# Autodesk Inventor assembly: FGR AL-2-PGN-plus-P 160,PGN-plus-P 160-2-AS-P1Aluminium86.5165110452001216049.500000000000000002
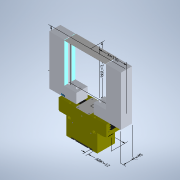
[picture p0: Inventor's stored thumbnail of the model, 180x180]
Saved by Autodesk Inventor 2021 (Build 250183000, 183)
## iProperties
Category: PARTsolutions
Company: SCHUNK
Created: 2025-07-30
Part Number: FGR AL-2-PGN-plus-P 160,PGN-plus-P 160-2-AS-P1Aluminium86.5165110452001216049.500000000000000002
Catalog Web Link: www.cadenas.de
Description: FGR-Customizable gripper fingers
Vendor: SCHUNK
Document SubType Name: Assembly
Designer: psAdmin
Manufacturer: SCHUNK
Mass: 2444.6 g
Surface Area: 3300.31 cm^2
Volume: 2444.6 cm^3
Density: 1 g/cm^3
Title: FGR AL-2-PGN-plus-P 160, 11045200SPANNKONT.
Author: Cadenas PARTsolutions
Comments: Customizable gripper fingers
PSOL_IDENT_0: {$CADENAS_DATA/23d-libs/schunk/greifsysteme/konfigurationen/system_baukasten/easy_finger/easy_finger
PSOL_IDENT_1: _asm_at.prj},511 {M=Nenngewinde},{VTYP=3D},{STYP=ASSTAB},{NB=FGR AL-2-PGN-plus-P 160,PGN-plus-P 160-
PSOL_IDENT_2: 2-AS-P1Aluminium86.5165110452001216049.500000000000000002},{LINA=FGR AL-2-PGN-plus-P 160, 11045200SP
PSOL_IDENT_3: ANNKONT.},{NN=FGR},{DATE=29.07.2025 14:42:42},{GEOMDATE=25.10.2024 10:48:57},{VERSION=},{LINEID=10},
PSOL_IDENT_4: {WBVAR=BR,BGVR,ASIS,SPANNKONT,CNSMAT,WAERMEBE,HUB,RH,X,Y,Z,DWS,ABK,GFL,GFT,PP,PW,RA,EFO,FASE1,FL1,FA
PSOL_IDENT_5: SE2,FL2,FASE3,FW3,FL3,FASE4,FW4,FL4,BM},{WBNUMERIC=HUB,RH,X,Y,Z,DWS,ABK,GFL,GFT,PP,PW,RA,EFO,FL1,FL2
PSOL_IDENT_6: ,FASE3,FW3,FL3,FW4,FL4,BM}  {NB=FGR AL-2-PGN-plus-P 160,PGN-plus-P 160-2-AS-P1Aluminium86.5165110452
PSOL_IDENT_7: 001216049.500000000000000002},{LINA=FGR AL-2-PGN-plus-P 160, 11045200SPANNKONT.},{KT=DUMMY},{NT=Kund
PSOL_IDENT_8: enspezifisch konfigurierbare Greiferfinger},{START=Geometriemodell 2},{VERSION=1},{VER=V1},{MATN=378
PSOL_IDENT_9: 6171200_fgr_gl_ia_v1},{XMLMATN=material|},{XMLMAT=AlZn55MgCu_EN-AW-7075_34365},{TYP=FGR AL-2-PGN-plu
PSOL_IDENT_10: s-P 160},{TYPX=PGN-plus-P 160},{TYPXMAT=AL},{TYPXX=PGN-plus-P 160},{BR=PGN-plus-P},{BG=160.0},{BGVR=
PSOL_IDENT_11: PGN-plus-P 160-2-AS-P},{BGVRX='PGN-plus-P 40','PGN-plus-P 40','PGN-plus-P 40-SD','PGN-plus-P 40-SD','
PSOL_IDENT_12: PGN-plus-P 40-K','PGN-plus-P 40-K','PGN-plus-P 40-V','PGN-plus-P 40-V','PGN-plus-P 40-P','PGN-plus-P
PSOL_IDENT_13: 40-P','PGN-plus-P 40-AS','PGN-plus-P 40-AS','PGN-plus-P 40-AS-SD','PGN-plus-P 40-AS-SD','PGN-plus-P
PSOL_IDENT_14: 40-AS-K','PGN-plus-P 40-AS-K','PGN-plus-P 40-AS-V','PGN-plus-P 40-AS-V','PGN-plus-P 40-AS-P','PGN-p
PSOL_IDENT_15: lus-P 40-AS-P','PGN-plus-P 40-IS','PGN-plus-P 40-IS','PGN-plus-P 40-IS-SD','PGN-plus-P 40-IS-SD','PG
PSOL_IDENT_16: N-plus-P 40-IS-K','PGN-plus-P 40-IS-K','PGN-plus-P 40-IS-V','PGN-plus-P 40-IS-V','PGN-plus-P 50-1','
PSOL_IDENT_17: PGN-plus-P 50-1','PGN-plus-P 50-1-SD','PGN-plus-P 50-1-SD','PGN-plus-P 50-1-K','PGN-plus-P 50-1-K','
PSOL_IDENT_18: PGN-plus-P 50-1-V','PGN-plus-P 50-1-V','PGN-plus-P 50-1-P','PGN-plus-P 50-1-P','PGN-plus-P 50-2','PG
PSOL_IDENT_19: N-plus-P 50-2','PGN-plus-P 50-2-SD','PGN-plus-P 50-2-SD','PGN-plus-P 50-2-K','PGN-plus-P 50-2-K','PG
PSOL_IDENT_20: N-plus-P 50-2-V','PGN-plus-P 50-2-V','PGN-plus-P 50-2-P','PGN-plus-P 50-2-P','PGN-plus-P 50-1-AS','P
PSOL_IDENT_21: GN-plus-P 50-1-AS','PGN-plus-P 50-1-AS-SD','PGN-plus-P 50-1-AS-SD','PGN-plus-P 50-1-AS-K','PGN-plus-
PSOL_IDENT_22: P 50-1-AS-K','PGN-plus-P 50-1-AS-V','PGN-plus-P 50-1-AS-V','PGN-plus-P 50-1-AS-P','PGN-plus-P 50-1-A
PSOL_IDENT_23: S-P','PGN-plus-P 50-2-AS','PGN-plus-P 50-2-AS','PGN-plus-P 50-2-AS-SD','PGN-plus-P 50-2-AS-SD','PGN-
PSOL_IDENT_24: plus-P 50-2-AS-K','PGN-plus-P 50-2-AS-K','PGN-plus-P 50-2-AS-V','PGN-plus-P 50-2-AS-V','PGN-plus-P 5
PSOL_IDENT_25: 0-2-AS-P','PGN-plus-P 50-2-AS-P','PGN-plus-P 50-1-IS','PGN-plus-P 50-1-IS','PGN-plus-P 50-1-IS-SD','
PSOL_IDENT_26: PGN-plus-P 50-1-IS-SD','PGN-plus-P 50-1-IS-K','PGN-plus-P 50-1-IS-K','PGN-plus-P 50-1-IS-V','PGN-plu
PSOL_IDENT_27: s-P 50-1-IS-V','PGN-plus-P 50-2-IS','PGN-plus-P 50-2-IS','PGN-plus-P 50-2-IS-SD','PGN-plus-P 50-2-IS
PSOL_IDENT_28: -SD','PGN-plus-P 50-2-IS-K','PGN-plus-P 50-2-IS-K','PGN-plus-P 50-2-IS-V','PGN-plus-P 50-2-IS-V','PG
PSOL_IDENT_29: N-plus-P 64-1','PGN-plus-P 64-1','PGN-plus-P 64-1-SD','PGN-plus-P 64-1-SD','PGN-plus-P 64-1-K','PGN-
PSOL_IDENT_30: plus-P 64-1-K','PGN-plus-P 64-1-V','PGN-plus-P 64-1-V','PGN-plus-P 64-1-P','PGN-plus-P 64-1-P','PGN-
PSOL_IDENT_31: plus-P 64-2','PGN-plus-P 64-2','PGN-plus-P 64-2-SD','PGN-plus-P 64-2-SD','PGN-plus-P 64-2-K','PGN-pl
PSOL_IDENT_32: us-P 64-2-K','PGN-plus-P 64-2-V','PGN-plus-P 64-2-V','PGN-plus-P 64-2-P','PGN-plus-P 64-2-P','PGN-pl
PSOL_IDENT_33: us-P 64-1-AS','PGN-plus-P 64-1-AS','PGN-plus-P 64-1-AS-SD','PGN-plus-P 64-1-AS-SD','PGN-plus-P 64-1-
PSOL_IDENT_34: AS-K','PGN-plus-P 64-1-AS-K','PGN-plus-P 64-1-AS-V','PGN-plus-P 64-1-AS-V','PGN-plus-P 64-1-AS-P','P
PSOL_IDENT_35: GN-plus-P 64-1-AS-P','PGN-plus-P 64-2-AS','PGN-plus-P 64-2-AS','PGN-plus-P 64-1-IS','PGN-plus-P 64-1
PSOL_IDENT_36: -IS','PGN-plus-P 64-1-IS-SD','PGN-plus-P 64-1-IS-SD','PGN-plus-P 64-1-IS-K','PGN-plus-P 64-1-IS-K','
PSOL_IDENT_37: PGN-plus-P 64-1-IS-V','PGN-plus-P 64-1-IS-V','PGN-plus-P 64-2-IS','PGN-plus-P 64-2-IS','PGN-plus-P 6
PSOL_IDENT_38: 4-2-IS-SD','PGN-plus-P 64-2-IS-SD','PGN-plus-P 64-2-IS-K','PGN-plus-P 64-2-IS-K','PGN-plus-P 64-2-V'
PSOL_IDENT_39: ,'PGN-plus-P 64-2-V','PGN-plus-P 80-1','PGN-plus-P 80-1','PGN-plus-P 80-1-SD','PGN-plus-P 80-1-SD','
PSOL_IDENT_40: PGN-plus-P 80-1-K','PGN-plus-P 80-1-K','PGN-plus-P 80-1-V','PGN-plus-P 80-1-V','PGN-plus-P 80-1-P','
PSOL_IDENT_41: PGN-plus-P 80-1-P','PGN-plus-P 80-2','PGN-plus-P 80-2','PGN-plus-P 80-2-SD','PGN-plus-P 80-2-SD','PG
PSOL_IDENT_42: N-plus-P 80-2-K','PGN-plus-P 80-2-K','PGN-plus-P 80-2-V','PGN-plus-P 80-2-V','PGN-plus-P 80-2-P','PG
PSOL_IDENT_43: N-plus-P 80-2-P','PGN-plus-P 80-1-AS','PGN-plus-P 80-1-AS','PGN-plus-P 80-1-AS-SD','PGN-plus-P 80-1-
PSOL_IDENT_44: AS-SD','PGN-plus-P 80-1-AS-K','PGN-plus-P 80-1-AS-K','PGN-plus-P 80-1-AS-V','PGN-plus-P 80-1-AS-V','
PSOL_IDENT_45: PGN-plus-P 80-1-AS-P','PGN-plus-P 80-1-AS-P','PGN-plus-P 80-2-AS','PGN-plus-P 80-2-AS','PGN-plus-P 8
PSOL_IDENT_46: 0-2-AS-SD', 'PGN-plus-P 80-2-AS-SD','PGN-plus-P 80-2-AS-K','PGN-plus-P 80-2-AS-K','PGN-plus-P 80-2-A
PSOL_IDENT_47: S-V','PGN-plus-P 80-2-AS-V','PGN-plus-P 80-2-AS-P','PGN-plus-P 80-2-AS-P','PGN-plus-P 80-1-IS','PGN-
PSOL_IDENT_48: plus-P 80-1-IS','PGN-plus-P 80-1-IS-SD','PGN-plus-P 80-1-IS-SD','PGN-plus-P 80-1-IS-K','PGN-plus-P 8
PSOL_IDENT_49: 0-1-IS-K','PGN-plus-P 80-1-IS-V','PGN-plus-P 80-1-IS-V','PGN-plus-P 80-2-IS','PGN-plus-P 80-2-IS','P
PSOL_IDENT_50: GN-plus-P 80-2-IS-SD','PGN-plus-P 80-2-IS-SD','PGN-plus-P 80-2-IS-K','PGN-plus-P 80-2-IS-K','PGN-plu
PSOL_IDENT_51: s-P 80-2-IS-V','PGN-plus-P 80-2-IS-V','PGN-plus-P 100-1','PGN-plus-P 100-1','PGN-plus-P 100-1-SD','P
PSOL_IDENT_52: GN-plus-P 100-1-SD','PGN-plus-P 100-1-K','PGN-plus-P 100-1-K','PGN-plus-P 100-1-V','PGN-plus-P 100-1
PSOL_IDENT_53: -V','PGN-plus-P 100-1-P','PGN-plus-P 100-1-P','PGN-plus-P 100-2','PGN-plus-P 100-2','PGN-plus-P 100-
PSOL_IDENT_54: 2-SD','PGN-plus-P 100-2-SD','PGN-plus-P 100-2-K','PGN-plus-P 100-2-K','PGN-plus-P 100-2-V','PGN-plus
PSOL_IDENT_55: -P 100-2-V','PGN-plus-P 100-2-P','PGN-plus-P 100-2-P','PGN-plus-P 100-1-AS','PGN-plus-P 100-1-AS','P
PSOL_IDENT_56: GN-plus-P 100-1-AS-SD','PGN-plus-P 100-1-AS-SD','PGN-plus-P 100-1-AS-K','PGN-plus-P 100-1-AS-K','PGN
PSOL_IDENT_57: -plus-P 100-1-AS-V','PGN-plus-P 100-1-AS-V','PGN-plus-P 100-1-AS-P','PGN-plus-P 100-1-AS-P','PGN-plu
PSOL_IDENT_58: s-P 100-2-AS','PGN-plus-P 100-2-AS','PGN-plus-P 100-2-AS-SD','PGN-plus-P 100-2-AS-SD','PGN-plus-P 10
PSOL_IDENT_59: 0-2-AS-K','PGN-plus-P 100-2-AS-K','PGN-plus-P 100-2-AS-V','PGN-plus-P 100-2-AS-V','PGN-plus-P 100-2-
PSOL_IDENT_60: AS-P','PGN-plus-P 100-2-AS-P','PGN-plus-P 100-1-IS','PGN-plus-P 100-1-IS','PGN-plus-P 100-1-IS-SD','
PSOL_IDENT_61: PGN-plus-P 100-1-IS-SD','PGN-plus-P 100-1-IS-K','PGN-plus-P 100-1-IS-K','PGN-plus-P 100-1-IS-V','PGN
PSOL_IDENT_62: -plus-P 100-1-IS-V','PGN-plus-P 100-2-IS','PGN-plus-P 100-2-IS','PGN-plus-P 100-2-IS-SD','PGN-plus-P
PSOL_IDENT_63: 100-2-IS-SD','PGN-plus-P 100-2-IS-K','PGN-plus-P 100-2-IS-K','PGN-plus-P 100-2-IS-V','PGN-plus-P 10
PSOL_IDENT_64: 0-2-IS-V','PGN-plus-P 125-1','PGN-plus-P 125-1','PGN-plus-P 125-1-SD','PGN-plus-P 125-1-SD','PGN-plu
PSOL_IDENT_65: s-P 125-1-K','PGN-plus-P 125-1-K','PGN-plus-P 125-1-V','PGN-plus-P 125-1-V','PGN-plus-P 125-1-P','PG
PSOL_IDENT_66: N-plus-P 125-1-P','PGN-plus-P 125-2','PGN-plus-P 125-2','PGN-plus-P 125-2-SD','PGN-plus-P 125-2-SD','
PSOL_IDENT_67: PGN-plus-P 125-2-K','PGN-plus-P 125-2-K','PGN-plus-P 125-2-V','PGN-plus-P 125-2-V','PGN-plus-P 125-2
PSOL_IDENT_68: -P','PGN-plus-P 125-2-P','PGN-plus-P 125-1-AS','PGN-plus-P 125-1-AS','PGN-plus-P 125-1-AS-SD','PGN-p
PSOL_IDENT_69: lus-P 125-1-AS-SD','PGN-plus-P 125-1-AS-K','PGN-plus-P 125-1-AS-K','PGN-plus-P 125-1-AS-V','PGN-plus
PSOL_IDENT_70: -P 125-1-AS-V','PGN-plus-P 125-1-AS-P','PGN-plus-P 125-1-AS-P','PGN-plus-P 125-2-AS','PGN-plus-P 125
PSOL_IDENT_71: -2-AS','PGN-plus-P 125-2-AS-SD','PGN-plus-P 125-2-AS-SD','PGN-plus-P 125-2-AS-K','PGN-plus-P 125-2-A
PSOL_IDENT_72: S-K','PGN-plus-P 125-2-AS-V','PGN-plus-P 125-2-AS-V','PGN-plus-P 125-2-AS-P','PGN-plus-P 125-2-AS-P'
PSOL_IDENT_73: ,'PGN-plus-P 125-1-IS','PGN-plus-P 125-1-IS','PGN-plus-P 125-1-IS-SD','PGN-plus-P 125-1-IS-SD','PGN-
PSOL_IDENT_74: plus-P 125-1-IS-K','PGN-plus-P 125-1-IS-K','PGN-plus-P 125-1-IS-V','PGN-plus-P 125-1-IS-V','PGN-plus
PSOL_IDENT_75: -P 125-2-IS','PGN-plus-P 125-2-IS','PGN-plus-P 125-2-IS-SD','PGN-plus-P 125-2-IS-SD','PGN-plus-P 125
PSOL_IDENT_76: -2-IS-K','PGN-plus-P 125-2-IS-K','PGN-plus-P 125-2-IS-V','PGN-plus-P 125-2-IS-V','PGN-plus-P 160-1','
PSOL_IDENT_77: PGN-plus-P 160-1','PGN-plus-P 160-1-SD','PGN-plus-P 160-1-SD','PGN-plus-P 160-1-K','PGN-plus-P 160-1
PSOL_IDENT_78: -K','PGN-plus-P 160-1-V','PGN-plus-P 160-1-V','PGN-plus-P 160-1-P','PGN-plus-P 160-1-P','PGN-plus-P
PSOL_IDENT_79: 160-2','PGN-plus-P 160-2','PGN-plus-P 160-2-SD','PGN-plus-P 160-2-SD','PGN-plus-P 160-2-K','PGN-plus
PSOL_IDENT_80: -P 160-2-K','PGN-plus-P 160-2-V','PGN-plus-P 160-2-V','PGN-plus-P 160-2-P','PGN-plus-P 160-2-P','PGN
PSOL_IDENT_81: -plus-P 160-1-AS','PGN-plus-P 160-1-AS','PGN-plus-P 160-1-AS-SD','PGN-plus-P 160-1-AS-SD','PGN-plus-
PSOL_IDENT_82: P 160-1-AS-K','PGN-plus-P 160-1-AS-K','PGN-plus-P 160-1-AS-V','PGN-plus-P 160-1-AS-V','PGN-plus-P 16
PSOL_IDENT_83: 0-1-AS-P','PGN-plus-P 160-1-AS-P','PGN-plus-P 160-2-AS','PGN-plus-P 160-2-AS','PGN-plus-P 160-2-AS-S
PSOL_IDENT_84: D','PGN-plus-P 160-2-AS-SD','PGN-plus-P 160-2-AS-K','PGN-plus-P 160-2-AS-K','PGN-plus-P 160-2-AS-V','
PSOL_IDENT_85: PGN-plus-P 160-2-AS-V','PGN-plus-P 160-2-AS-P','PGN-plus-P 160-2-AS-P','PGN-plus-P 160-1-IS','PGN-pl
PSOL_IDENT_86: us-P 160-1-IS','PGN-plus-P 160-1-IS-SD','PGN-plus-P 160-1-IS-SD','PGN-plus-P 160-1-IS-K','PGN-plus-P
PSOL_IDENT_87: 160-1-IS-K','PGN-plus-P 160-1-IS-V','PGN-plus-P 160-1-IS-V','PGN-plus-P 160-2-IS','PGN-plus-P 160-2
PSOL_IDENT_88: -IS','PGN-plus-P 160-2-IS-SD','PGN-plus-P 160-2-IS-SD','PGN-plus-P 160-2-IS-K','PGN-plus-P 160-2-IS-
PSOL_IDENT_89: K','PGN-plus-P 160-2-IS-V','PGN-plus-P 160-2-IS-V','PGN-plus-P 200-1','PGN-plus-P 200-1','PGN-plus-P
PSOL_IDENT_90: 200-1-SD','PGN-plus-P 200-1-SD','PGN-plus-P 200-1-K','PGN-plus-P 200-1-K','PGN-plus-P 200-1-V','PGN
PSOL_IDENT_91: -plus-P 200-1-V','PGN-plus-P 200-1-P','PGN-plus-P 200-1-P','PGN-plus-P 200-2','PGN-plus-P 200-2','PG
PSOL_IDENT_92: N-plus-P 200-2-SD','PGN-plus-P 200-2-SD','PGN-plus-P 200-2-K','PGN-plus-P 200-2-K','PGN-plus-P 200-2
PSOL_IDENT_93: -V','PGN-plus-P 200-2-V','PGN-plus-P 200-2-P','PGN-plus-P 200-2-P','PGN-plus-P 200-1-AS','PGN-plus-P
PSOL_IDENT_94: 200-1-AS','PGN-plus-P 200-1-AS-SD','PGN-plus-P 200-1-AS-SD','PGN-plus-P 200-1-AS-K','PGN-plus-P 200
PSOL_IDENT_95: -1-AS-K','PGN-plus-P 200-1-AS-V','PGN-plus-P 200-1-AS-V','PGN-plus-P 200-1-AS-P','PGN-plus-P 200-1-A
PSOL_IDENT_96: S-P','PGN-plus-P 200-2-AS','PGN-plus-P 200-2-AS','PGN-plus-P 200-2-AS-SD','PGN-plus-P 200-2-AS-SD','
PSOL_IDENT_97: PGN-plus-P 200-2-AS-K','PGN-plus-P 200-2-AS-K','PGN-plus-P 200-2-AS-V','PGN-plus-P 200-2-AS-V','PGN-
PSOL_IDENT_98: plus-P 200-2-AS-P','PGN-plus-P 200-2-AS-P','PGN-plus-P 200-1-IS','PGN-plus-P 200-1-IS','PGN-plus-P 2
PSOL_IDENT_99: 00-1-IS-SD','PGN-plus-P 200-1-IS-SD','PGN-plus-P 200-1-IS-K','PGN-plus-P 200-1-IS-K','PGN-plus-P 200
PSOL_IDENT_100: -1-IS-V','PGN-plus-P 200-1-IS-V','PGN-plus-P 200-2-IS','PGN-plus-P 200-2-IS','PGN-plus-P 200-2-IS-SD'
PSOL_IDENT_101: ,'PGN-plus-P 200-2-IS-SD','PGN-plus-P 200-2-IS-K','PGN-plus-P 200-2-IS-K','PGN-plus-P 200-2-IS-V','P
PSOL_IDENT_102: GN-plus-P 200-2-IS-V','PGN-plus-P 240-1','PGN-plus-P 240-1','PGN-plus-P 240-1-SD','PGN-plus-P 240-1-
PSOL_IDENT_103: SD','PGN-plus-P 240-1-K','PGN-plus-P 240-1-K','PGN-plus-P 240-1-V','PGN-plus-P 240-1-V','PGN-plus-P
PSOL_IDENT_104: 240-1-P','PGN-plus-P 240-1-P','PGN-plus-P 240-2','PGN-plus-P 240-2','PGN-plus-P 240-2-SD','PGN-plus-
PSOL_IDENT_105: P 240-2-SD','PGN-plus-P 240-2-K','PGN-plus-P 240-2-K','PGN-plus-P 240-2-V','PGN-plus-P 240-2-V','PGN
PSOL_IDENT_106: -plus-P 240-2-P','PGN-plus-P 240-2-P', 'PGN-plus-P 240-1-AS','PGN-plus-P 240-1-AS','PGN-plus-P 240-1
PSOL_IDENT_107: -AS-SD','PGN-plus-P 240-1-AS-SD','PGN-plus-P 240-1-AS-K','PGN-plus-P 240-1-AS-K','PGN-plus-P 240-1-A
PSOL_IDENT_108: S-V','PGN-plus-P 240-1-AS-V','PGN-plus-P 240-1-AS-P','PGN-plus-P 240-1-AS-P', 'PGN-plus-P 240-2-AS','
PSOL_IDENT_109: PGN-plus-P 240-2-AS','PGN-plus-P 240-2-AS-SD','PGN-plus-P 240-2-AS-SD','PGN-plus-P 240-2-AS-K','PGN-
PSOL_IDENT_110: plus-P 240-2-AS-K','PGN-plus-P 240-2-AS-V','PGN-plus-P 240-2-AS-V','PGN-plus-P 240-2-AS-P','PGN-plus
PSOL_IDENT_111: -P 240-2-AS-P', 'PGN-plus-P 240-1-IS','PGN-plus-P 240-1-IS','PGN-plus-P 240-1-IS-SD','PGN-plus-P 240
PSOL_IDENT_112: -1-IS-SD','PGN-plus-P 240-1-IS-K','PGN-plus-P 240-1-IS-K','PGN-plus-P 240-1-IS-V','PGN-plus-P 240-1-
PSOL_IDENT_113: IS-V', 'PGN-plus-P 240-2-IS','PGN-plus-P 240-2-IS','PGN-plus-P 240-2-IS-SD','PGN-plus-P 240-2-IS-SD'
PSOL_IDENT_114: ,'PGN-plus-P 240-2-IS-K','PGN-plus-P 240-2-IS-K','PGN-plus-P 240-2-IS-V','PGN-plus-P 240-2-IS-V','PG
PSOL_IDENT_115: N-plus-P 300-1','PGN-plus-P 300-1','PGN-plus-P 300-1-SD','PGN-plus-P 300-1-SD','PGN-plus-P 300-1-K','
PSOL_IDENT_116: PGN-plus-P 300-1-K','PGN-plus-P 300-1-V','PGN-plus-P 300-1-V','PGN-plus-P 300-1-P','PGN-plus-P 300-1
PSOL_IDENT_117: -P','PGN-plus-P 300-2','PGN-plus-P 300-2','PGN-plus-P 300-2-SD','PGN-plus-P 300-2-SD','PGN-plus-P 30
PSOL_IDENT_118: 0-2-K','PGN-plus-P 300-2-K','PGN-plus-P 300-2-V','PGN-plus-P 300-2-V','PGN-plus-P 300-2-P','PGN-plus
PSOL_IDENT_119: -P 300-2-P', 'PGN-plus-P 300-1-AS','PGN-plus-P 300-1-AS','PGN-plus-P 300-1-AS-SD','PGN-plus-P 300-1-
PSOL_IDENT_120: AS-SD','PGN-plus-P 300-1-AS-K','PGN-plus-P 300-1-AS-K','PGN-plus-P 300-1-AS-V','PGN-plus-P 300-1-AS-
PSOL_IDENT_121: V','PGN-plus-P 300-1-AS-P','PGN-plus-P 300-1-AS-P', 'PGN-plus-P 300-2-AS','PGN-plus-P 300-2-AS','PGN
PSOL_IDENT_122: -plus-P 300-2-AS-SD','PGN-plus-P 300-2-AS-SD','PGN-plus-P 300-2-AS-K','PGN-plus-P 300-2-AS-K','PGN-p
PSOL_IDENT_123: lus-P 300-2-AS-V','PGN-plus-P 300-2-AS-V','PGN-plus-P 300-2-AS-P','PGN-plus-P 300-2-AS-P', 'PGN-plus
PSOL_IDENT_124: -P 300-1-IS','PGN-plus-P 300-1-IS','PGN-plus-P 300-1-IS-SD','PGN-plus-P 300-1-IS-SD','PGN-plus-P 300
PSOL_IDENT_125: -1-IS-K','PGN-plus-P 300-1-IS-K','PGN-plus-P 300-1-IS-V','PGN-plus-P 300-1-IS-V', 'PGN-plus-P 300-2-
PSOL_IDENT_126: IS','PGN-plus-P 300-2-IS','PGN-plus-P 300-2-IS-SD','PGN-plus-P 300-2-IS-SD','PGN-plus-P 300-2-IS-K','
PSOL_IDENT_127: PGN-plus-P 300-2-IS-K','PGN-plus-P 300-2-IS-V','PGN-plus-P 300-2-IS-V','PGN-plus-P 380-1','PGN-plus-
PSOL_IDENT_128: P 380-1','PGN-plus-P 380-1-SD','PGN-plus-P 380-1-SD','PGN-plus-P 380-1-K','PGN-plus-P 380-1-K','PGN-
PSOL_IDENT_129: plus-P 380-1-V','PGN-plus-P 380-1-V','PGN-plus-P 380-1-P','PGN-plus-P 380-1-P','PGN-plus-P 380-2','P
PSOL_IDENT_130: GN-plus-P 380-2','PGN-plus-P 380-2-SD','PGN-plus-P 380-2-SD','PGN-plus-P 380-2-K','PGN-plus-P 380-2-
PSOL_IDENT_131: K','PGN-plus-P 380-2-V','PGN-plus-P 380-2-V','PGN-plus-P 380-2-P','PGN-plus-P 380-2-P', 'PGN-plus-P
PSOL_IDENT_132: 380-1-AS','PGN-plus-P 380-1-AS','PGN-plus-P 380-1-AS-SD','PGN-plus-P 380-1-AS-SD','PGN-plus-P 380-1-
PSOL_IDENT_133: AS-K','PGN-plus-P 380-1-AS-K','PGN-plus-P 380-1-AS-V','PGN-plus-P 380-1-AS-V','PGN-plus-P 380-1-AS-P'
PSOL_IDENT_134: ,'PGN-plus-P 380-1-AS-P', 'PGN-plus-P 380-2-AS','PGN-plus-P 380-2-AS','PGN-plus-P 380-2-AS-SD','PGN-
PSOL_IDENT_135: plus-P 380-2-AS-SD','PGN-plus-P 380-2-AS-K','PGN-plus-P 380-2-AS-K','PGN-plus-P 380-2-AS-V','PGN-plu
PSOL_IDENT_136: s-P 380-2-AS-V','PGN-plus-P 380-2-AS-P','PGN-plus-P 380-2-AS-P', 'PGN-plus-P 380-1-IS','PGN-plus-P 3
PSOL_IDENT_137: 80-1-IS','PGN-plus-P 380-1-IS-SD','PGN-plus-P 380-1-IS-SD','PGN-plus-P 380-1-IS-K','PGN-plus-P 380-1
PSOL_IDENT_138: -IS-K','PGN-plus-P 380-1-IS-V','PGN-plus-P 380-1-IS-V', 'PGN-plus-P 380-2-IS','PGN-plus-P 380-2-IS','
PSOL_IDENT_139: PGN-plus-P 380-2-IS-SD','PGN-plus-P 380-2-IS-SD','PGN-plus-P 380-2-IS-K','PGN-plus-P 380-2-IS-K','PG
PSOL_IDENT_140: N-plus-P 380-2-IS-V','PGN-plus-P 380-2-IS-V'},{BGVRZ=116.800},{BGVRXX=77.0},{ZBAX=109.0},{IDNR=13176
PSOL_IDENT_141: 60},{ASIS=1},{ASISX=<'1','Außengreifen','aussengreifen.png'>,'2','Innnengreifen','innengreifen.png'}
PSOL_IDENT_142: ,{ASISXX=AS},{SPANNKONT=2},{SPANNKONTX='1', 'Gerader Greiferfinger', 'startmodell_1.png', '2' , 'Gre
PSOL_IDENT_143: iferfinger mit nach innen abgesetzter Greiffläche', 'startmodell_2.png', '3' , 'Greiferfinger mit na
PSOL_IDENT_144: ch außen abgesetzter Greiffläche', 'startmodell_3.png', '4' , 'Greiferfinger mit nach innen abgesetz
PSOL_IDENT_145: ter und abgerundeter Greiffläche', 'startmodell_4.png', '5' , 'Greiferfinger mit nach außen abgesetz
PSOL_IDENT_146: ter und abgerundeter Greiffläche', 'startmodell_5.png', '6' , 'Greiferfinger mit nach innen abgesetz
PSOL_IDENT_147: ter Greiffläche und vertikalem Prisma', 'startmodell_6.png','8' , 'Greiferfinger mit horizontalem Pr
PSOL_IDENT_148: isma', 'startmodell_8.png'},{CNSMAT=Aluminium},{WAERMEBE=},{WAERMEBEX='',''},{SAPWAERMEBE=10},{HUB=8
PSOL_IDENT_149: .0},{HMAX=8.0},{RH=6.5},{HMAXX=8.0},{RHB=2.0},{GFM=38.50},{GFMAS=38.50},{GFMIS=70.50},{X=110.0},{XMI
PSOL_IDENT_150: N=56.0},{XMAX=113.0},{XTEST=[56:113/0.1]},{MAXX=113.0},{Y=45.0},{YMIN=27.0},{YMAX=60.0},{MAXY=60.0},
PSOL_IDENT_151: {Z=200.0},{ZMIN=32.0},{ZMAX=200.0},{ZMAXX=100.0},{MAXZ=200.0},{DWS=165.0},{DWSX=[68:222]},{DWSMIN=68
PSOL_IDENT_152: .000},{DWSMAX=222.000},{DWSMAXX=111.0},{DWSXX=1.000},{DWSZ=1.000},{DWS1V=70.0},{DWS1H=110.0},{DWS2V=
PSOL_IDENT_153: 134.0},{GWI=1.0},{ABK=12.00},{ABKMIN=12.00},{ABKMAX=37.50},{GFL=160.0},{GFLX=[1:169.4]},{GFLMIN=1.00
PSOL_IDENT_154: },{GFLMAX=169.40},{GFT=49.50},{GFTX=[49.5:49.5/0.1]},{GFTMIN=49.50},{GFTMINTH=-217577236067824.12},{
PSOL_IDENT_155: GFTMAX=49.50},{GFT1V=2.00},{GFT1H=22.00},{GFT2V=34.00},{GFT2H=54.00},{SKS=10.6},{PP=0.0},{PPX=[0]},{
PSOL_IDENT_156: PPMIN=0.0},{PPMAX=0.0},{PUK=0.00},{PUKZ=88.50},{PUKX=0.00},{PW=0.0},{PWX=[0]},{PWMIN=120},{PWMAX=120
PSOL_IDENT_157: },{PWTH=120.0},{PWTHX=180.000},{ALPHA=0.000},{RA=0.0},{RAX=[0]},{RAMIN=1.0},{RAMAX=44},{EFO=0.0},{EF
PSOL_IDENT_158: OX=[0]},{EFOMAX=0.10},{FASE1=0},{FASE1X='0','ohne Fase 1','kein_bild.png','1','mit Fase 1','fase_1.p
PSOL_IDENT_159: ng'},{FW1=0.0},{FL1=0.0},{FL1MIN=0.0},{FL1MAX=0.0},{FASE2=0},{FASE2X='0','ohne Fase 2','kein_bild.pn
PSOL_IDENT_160: g','1','mit Fase 2','fase_2.png'},{FW2=0.0},{FL2=0.0},{FL2MIN=0.0},{FL2MAX=0.0},{FASE3=0},{FW3=0.0},
PSOL_IDENT_161: {FW3MIN=0.0},{FW3MAX=0.0},{FL3=0.0},{FL3MIN=0.0},{FL3MAX=0.00},{FASE4=0},{FASE4X='0','ohne Fase 4','
PSOL_IDENT_162: kein_bild.png','1','mit Fase 4','fase_4_glatt.png'},{FW4=0.0},{FW4MIN=0.0},{FW4MAX=0.0},{FL4=0.0},{F
PSOL_IDENT_163: L4MIN=0.0},{FL4MAX=0.00},{ROH=1.457},{DICHTE=2.71},{ZULFM=3.800},{VALFM=true},{VOL=537767.200},{VFAS
PSOL_IDENT_164: E1=0.00},{VFASE2=0.00},{VFASE3=0.00},{VFASE4=0.00},{GFTXX=2.00},{STX1=20.00},{STX2=20.00},{EST=17.0}
PSOL_IDENT_165: ,{AB=32.0},{ZD=14.0},{ZT=4.0},{DB=11.0},{SD=18.0},{ST=20.00},{RI=8.2},{L=6.500},{LX=-31.000},{L1=1.0
PSOL_IDENT_166: 00},{L1X=-0.000},{L2=1.000},{LA=82.500},{GANS=M10},{PBO=11.0},{DPB=11.00},{RPO=3},{AQB=2.8},{SCHT=0.
PSOL_IDENT_167: 75},{SCHL=17.40},{SCHH=6.40},{SCHP=5.00},{TYPALU=3.00},{SCHGD=10.0},{SCHGL=35.0},{LZ=5 Werktage},{SA
PSOL_IDENT_168: PLZ=5},{VK=272.00},{VKB=226.11},{VKZ=33.92},{VKX=11.31},{VKP=0.00},{VKW=0.00},{ZX=200.0},{ZXX=100.0}
PSOL_IDENT_169: ,{XX=113.0},{XXX=56.5},{SPERR=0.00},{WC=3786171200_fgr_gl_ia_v1.prt},{MN=3786171200_FGR_GL_IA_V1},{X
PSOL_IDENT_170: MLX=dim|15},{XMLY=dim|14},{XMLZ=dim|13},{XMLAB=dim|35},{XMLABK=dim|71},{XMLFL1=dim|188},{XMLFL2=dim|
PSOL_IDENT_171: 151},{XMLFL3=dim|272},{XMLFW3=dim|274},{XMLFL4=dim|212},{XMLFW4=dim|211},{XMLGFL=dim|70},{XMLGFT=dim
PSOL_IDENT_172: |68},{XMLRA=},{XMLRI=},{XMLPW=},{XMLDWS=para|DWS},{XMLGFM=para|GFM},{XMLRH=},{XMLEFO=},{XMLPP=},{XML
PSOL_IDENT_173: ASIS=para|ASIS},{XMLVER=para|1|VER},{ANZ=2},{SG3D=8.0},{BM=2},{ZBUEGU=0},{PPATH=easy_finger_asmsbl.p
PSOL_IDENT_174: rj}
NB: FGR AL-2-PGN-plus-P 160,PGN-plus-P 160-2-AS-P1Aluminium86.5165110452001216049.500000000000000002
NN: FGR
NT: Customizable gripper fingers
NBSYN: $TYP.,$BGVR.$ASIS.$CNSMAT.$WAERMEBE.$HUB.$RH.$DWS.$X.$Y.$Z.$ABK.$GFL.$GFT.$PP.$PW.$RA.$EFO.$FASE1.$FW1.$FL1.$FASE2.$FW2.$FL2.$FASE3.$FW3.$FL3.$FASE4.$FW4.$FL4.$BM.
LINA: FGR AL-2-PGN-plus-P 160, 11045200SPANNKONT.
CATALOG: SCHUNK
BR: PGN-plus-P
BGVR: PGN-plus-P 160-2-AS-P
ASIS: O.D. gripping
SPANNKONT: Gripper finger with inwardly stepped gripping surface
CNSMAT: Aluminum AlZnMgCu1,5
HUB: 8
RH: 6.5
X: 110
Y: 45
Z: 200
DWS: 165
ABK: 12
GFL: 160
PP: 0
PW: 0
RA: 0
EFO: 0
FASE1: without chamfer 1
FL1: 0
FASE2: without chamfer 2
FL2: 0
FASE3: without chamfer 3
FW3: 0
FL3: 0
FASE4: without chamfer 4
FW4: 0
FL4: 0
ZULFM: 3.8
SUPPLIER: SCHUNK
ARTICLENO: FGR AL-2-PGN-plus-P 160,PGN-plus-P 160-2-AS-P1Aluminium86.5165110452001216049.500000000000000002
BOMINFO: FGR AL-2-PGN-plus-P 160, 11045200SPANNKONT.
CREATOR: CADENAS GmbH
## Documents named in this file (13)
- e:\temp\worker_COMMON_76\temp\tmp_5144_58_B99Yr\format_0\FGR AL-2-PGN-plus-P 160,PGN-plus-P 160-2-AS-P1Aluminium86_5165110452001216049_500000000000000002.iam
- e:\temp\worker_COMMON_76\temp\tmp_5144_58_B99Yr\format_0\SCHUNK-5524256 Gehaeuse-PGN-plus-P 160-GKS.ipt
- e:\temp\worker_COMMON_76\temp\tmp_5144_58_B99Yr\format_0\SCHUNK-5524251 Abdeckblech-PGN-plus-P 160.ipt
- e:\temp\worker_COMMON_76\temp\tmp_5144_58_B99Yr\format_0\SCHUNK-5524250 Deckel-PGN-plus-P 160.ipt
- e:\temp\worker_COMMON_76\temp\tmp_5144_58_B99Yr\format_0\SCHUNK-9949504 limit stop for MMS-P.ipt
- e:\temp\worker_COMMON_76\temp\tmp_5144_58_B99Yr\format_0\SCHUNK-9957615 Typenschild 16x64x0_3.ipt
- e:\temp\worker_COMMON_76\temp\tmp_5144_58_B99Yr\format_0\SCHUNK-5503506 Halter fuer NHS KL03.ipt
- e:\temp\worker_COMMON_76\temp\tmp_5144_58_B99Yr\format_0\SCHUNK---Grundbacke PGN-plus-P 160-2-P.ipt
- e:\temp\worker_COMMON_76\temp\tmp_5144_58_B99Yr\format_0\SCHUNK-9951430 Zentrierhuelse PGN-plus.ipt
- e:\temp\worker_COMMON_76\temp\tmp_5144_58_B99Yr\format_0\FGR AL-2-PGN-plus-P 160,PGN-plus-P 160-2-AS-P81110452001216049_51650000000000000000Aluminium6_5.ipt
- e:\temp\worker_COMMON_76\temp\tmp_5144_58_B99Yr\format_0\SCHUNK-9954530 Typenschild 6x17x0_3.ipt
- e:\temp\worker_COMMON_76\temp\tmp_5144_58_B99Yr\format_0\Slotted head cap screw ISO 4762 - M10x35.ipt
- e:\temp\worker_COMMON_76\temp\tmp_5144_58_B99Yr\format_0\FGR AL-2-PGN-plus-P 160 WKST,PGN-plus-P 160-2-AS-P18Aluminium6_5110452001216049_51650000000000000000.ipt
## Components (22 placed, 12 different names)
1. SCHUNK-5524256 Gehaeuse-PGN-plus-P 160-GKS:1 — adb_XY@1 <-> einbau_XY@2, adb_Z@1 <-> einbau_Z@2, adb_YZ@1 <-> einbau_YZ@2, dec_XY@1 <-> einbau_XY@3, dec_Z@1 <-> einbau_Z@3, dec_YZ@1 <-> einbau_YZ@3, ANS_1_XY@1 <-> ans_mms_p_XY@4, ANS_1_Z@1 <-> ans_mms_p_Z@4, ANS_1_YZ@1 <-> ans_mms_p_YZ@4, Typ_XY@1 <-> aluschild_XY@5, Typ_Z@1 <-> aluschild_Z@5, Typ_YZ@1 <-> aluschild_YZ@5, klh_2_XY@1 <-> klh_80_XY@6, klh_2_Z@1 <-> klh_80_Z@6, klh_2_YZ@1 <-> klh_80_YZ@6, klh_3_XY@1 <-> klh_80_XY@7, klh_3_Z@1 <-> klh_80_Z@7, klh_3_YZ@1 <-> klh_80_YZ@7
2. SCHUNK-5524251 Abdeckblech-PGN-plus-P 160:1 — adb_XY@1 <-> einbau_XY@2, adb_Z@1 <-> einbau_Z@2, adb_YZ@1 <-> einbau_YZ@2
3. SCHUNK-5524250 Deckel-PGN-plus-P 160:1 — dec_XY@1 <-> einbau_XY@3, dec_Z@1 <-> einbau_Z@3, dec_YZ@1 <-> einbau_YZ@3
4. SCHUNK-9949504 limit stop for MMS-P:1 — ANS_1_XY@1 <-> ans_mms_p_XY@4, ANS_1_Z@1 <-> ans_mms_p_Z@4, ANS_1_YZ@1 <-> ans_mms_p_YZ@4
5. SCHUNK-9957615 Typenschild 16x64x0_3:1 — Typ_XY@1 <-> aluschild_XY@5, Typ_Z@1 <-> aluschild_Z@5, Typ_YZ@1 <-> aluschild_YZ@5
6. SCHUNK-5503506 Halter fuer NHS KL03:1 — klh_2_XY@1 <-> klh_80_XY@6, klh_2_Z@1 <-> klh_80_Z@6, klh_2_YZ@1 <-> klh_80_YZ@6
7. SCHUNK-5503506 Halter fuer NHS KL03:2 — klh_3_XY@1 <-> klh_80_XY@7, klh_3_Z@1 <-> klh_80_Z@7, klh_3_YZ@1 <-> klh_80_YZ@7
8. SCHUNK---Grundbacke PGN-plus-P 160-2-P:1 — zhu1_XY@8 <-> gba_XY@9, zhu1_Z@8 <-> gba_Z@9, zhu1_YZ@8 <-> gba_YZ@9, zhu2_XY@8 <-> gba_XY@10, zhu2_Z@8 <-> gba_Z@10, zhu2_YZ@8 <-> gba_YZ@10
9. SCHUNK-9951430 Zentrierhuelse PGN-plus:1 — zhu1_XY@8 <-> gba_XY@9, zhu1_Z@8 <-> gba_Z@9, zhu1_YZ@8 <-> gba_YZ@9
10. SCHUNK-9951430 Zentrierhuelse PGN-plus:2 — zhu2_XY@8 <-> gba_XY@10, zhu2_Z@8 <-> gba_Z@10, zhu2_YZ@8 <-> gba_YZ@10
11. SCHUNK---Grundbacke PGN-plus-P 160-2-P:2 — zhu1_XY@11 <-> gba_XY@12, zhu1_Z@11 <-> gba_Z@12, zhu1_YZ@11 <-> gba_YZ@12, zhu2_XY@11 <-> gba_XY@13, zhu2_Z@11 <-> gba_Z@13, zhu2_YZ@11 <-> gba_YZ@13
12. SCHUNK-9951430 Zentrierhuelse PGN-plus:3 — zhu1_XY@11 <-> gba_XY@12, zhu1_Z@11 <-> gba_Z@12, zhu1_YZ@11 <-> gba_YZ@12
13. SCHUNK-9951430 Zentrierhuelse PGN-plus:4 — zhu2_XY@11 <-> gba_XY@13, zhu2_Z@11 <-> gba_Z@13, zhu2_YZ@11 <-> gba_YZ@13
14. FGR AL-2-PGN-plus-P 160,PGN-plus-P 160-2-AS-P81110452001216049_51650000000000000000Aluminium6_5:1 — IP_ALU_XY@14 <-> aluschild_XY@15, IP_ALU_Z@14 <-> aluschild_Z@15, IP_ALU_YZ@14 <-> aluschild_YZ@15, IP_SCH_1_XY@14 <-> IP1_XY@16, IP_SCH_1_Z@14 <-> IP1_Z@16, IP_SCH_1_YZ@14 <-> IP1_YZ@16, IP_SCH_2_XY@14 <-> IP1_XY@17, IP_SCH_2_Z@14 <-> IP1_Z@17, IP_SCH_2_YZ@14 <-> IP1_YZ@17
15. SCHUNK-9954530 Typenschild 6x17x0_3:1 — IP_ALU_XY@14 <-> aluschild_XY@15, IP_ALU_Z@14 <-> aluschild_Z@15, IP_ALU_YZ@14 <-> aluschild_YZ@15
16. Slotted head cap screw ISO 4762 - M10x35:1 — IP_SCH_1_XY@14 <-> IP1_XY@16, IP_SCH_1_Z@14 <-> IP1_Z@16, IP_SCH_1_YZ@14 <-> IP1_YZ@16
17. Slotted head cap screw ISO 4762 - M10x35:2 — IP_SCH_2_XY@14 <-> IP1_XY@17, IP_SCH_2_Z@14 <-> IP1_Z@17, IP_SCH_2_YZ@14 <-> IP1_YZ@17
18. FGR AL-2-PGN-plus-P 160,PGN-plus-P 160-2-AS-P81110452001216049_51650000000000000000Aluminium6_5:2 — IP_ALU_XY@18 <-> aluschild_XY@19, IP_ALU_Z@18 <-> aluschild_Z@19, IP_ALU_YZ@18 <-> aluschild_YZ@19, IP_SCH_1_XY@18 <-> IP1_XY@20, IP_SCH_1_Z@18 <-> IP1_Z@20, IP_SCH_1_YZ@18 <-> IP1_YZ@20, IP_SCH_2_XY@18 <-> IP1_XY@21, IP_SCH_2_Z@18 <-> IP1_Z@21, IP_SCH_2_YZ@18 <-> IP1_YZ@21
19. SCHUNK-9954530 Typenschild 6x17x0_3:2 — IP_ALU_XY@18 <-> aluschild_XY@19, IP_ALU_Z@18 <-> aluschild_Z@19, IP_ALU_YZ@18 <-> aluschild_YZ@19
20. Slotted head cap screw ISO 4762 - M10x35:3 — IP_SCH_1_XY@18 <-> IP1_XY@20, IP_SCH_1_Z@18 <-> IP1_Z@20, IP_SCH_1_YZ@18 <-> IP1_YZ@20
21. Slotted head cap screw ISO 4762 - M10x35:4 — IP_SCH_2_XY@18 <-> IP1_XY@21, IP_SCH_2_Z@18 <-> IP1_Z@21, IP_SCH_2_YZ@18 <-> IP1_YZ@21
22. FGR AL-2-PGN-plus-P 160 WKST,PGN-plus-P 160-2-AS-P18Aluminium6_5110452001216049_51650000000000000000:1
## Relationships (48: Mate 29, Angle 16, Flush 3)
- adb_XY@1 <-> einbau_XY@2 [Flush]: SCHUNK-5524256 Gehaeuse-PGN-plus-P 160-GKS:1 ↔ SCHUNK-5524251 Abdeckblech-PGN-plus-P 160:1
- adb_Z@1 <-> einbau_Z@2 [Mate]: SCHUNK-5524256 Gehaeuse-PGN-plus-P 160-GKS:1 ↔ SCHUNK-5524251 Abdeckblech-PGN-plus-P 160:1
- adb_YZ@1 <-> einbau_YZ@2 [Angle] (90 deg): SCHUNK-5524256 Gehaeuse-PGN-plus-P 160-GKS:1 ↔ SCHUNK-5524251 Abdeckblech-PGN-plus-P 160:1
- dec_XY@1 <-> einbau_XY@3 [Mate]: SCHUNK-5524256 Gehaeuse-PGN-plus-P 160-GKS:1 ↔ SCHUNK-5524250 Deckel-PGN-plus-P 160:1
- dec_Z@1 <-> einbau_Z@3 [Mate]: SCHUNK-5524256 Gehaeuse-PGN-plus-P 160-GKS:1 ↔ SCHUNK-5524250 Deckel-PGN-plus-P 160:1
- dec_YZ@1 <-> einbau_YZ@3 [Angle] (180 deg): SCHUNK-5524256 Gehaeuse-PGN-plus-P 160-GKS:1 ↔ SCHUNK-5524250 Deckel-PGN-plus-P 160:1
- ANS_1_XY@1 <-> ans_mms_p_XY@4 [Mate] (36 mm): SCHUNK-5524256 Gehaeuse-PGN-plus-P 160-GKS:1 ↔ SCHUNK-9949504 limit stop for MMS-P:1
- ANS_1_Z@1 <-> ans_mms_p_Z@4 [Mate]: SCHUNK-5524256 Gehaeuse-PGN-plus-P 160-GKS:1 ↔ SCHUNK-9949504 limit stop for MMS-P:1
- ANS_1_YZ@1 <-> ans_mms_p_YZ@4 [Angle] (0 deg): SCHUNK-5524256 Gehaeuse-PGN-plus-P 160-GKS:1 ↔ SCHUNK-9949504 limit stop for MMS-P:1
- Typ_XY@1 <-> aluschild_XY@5 [Flush]: SCHUNK-5524256 Gehaeuse-PGN-plus-P 160-GKS:1 ↔ SCHUNK-9957615 Typenschild 16x64x0_3:1
- Typ_Z@1 <-> aluschild_Z@5 [Mate]: SCHUNK-5524256 Gehaeuse-PGN-plus-P 160-GKS:1 ↔ SCHUNK-9957615 Typenschild 16x64x0_3:1
- Typ_YZ@1 <-> aluschild_YZ@5 [Angle] (180 deg): SCHUNK-5524256 Gehaeuse-PGN-plus-P 160-GKS:1 ↔ SCHUNK-9957615 Typenschild 16x64x0_3:1
- klh_2_XY@1 <-> klh_80_XY@6 [Flush]: SCHUNK-5524256 Gehaeuse-PGN-plus-P 160-GKS:1 ↔ SCHUNK-5503506 Halter fuer NHS KL03:1
- klh_2_Z@1 <-> klh_80_Z@6 [Mate]: SCHUNK-5524256 Gehaeuse-PGN-plus-P 160-GKS:1 ↔ SCHUNK-5503506 Halter fuer NHS KL03:1
- klh_2_YZ@1 <-> klh_80_YZ@6 [Angle] (0 deg): SCHUNK-5524256 Gehaeuse-PGN-plus-P 160-GKS:1 ↔ SCHUNK-5503506 Halter fuer NHS KL03:1
- klh_3_XY@1 <-> klh_80_XY@7 [Mate]: SCHUNK-5524256 Gehaeuse-PGN-plus-P 160-GKS:1 ↔ SCHUNK-5503506 Halter fuer NHS KL03:2
- klh_3_Z@1 <-> klh_80_Z@7 [Mate]: SCHUNK-5524256 Gehaeuse-PGN-plus-P 160-GKS:1 ↔ SCHUNK-5503506 Halter fuer NHS KL03:2
- klh_3_YZ@1 <-> klh_80_YZ@7 [Angle] (0 deg): SCHUNK-5524256 Gehaeuse-PGN-plus-P 160-GKS:1 ↔ SCHUNK-5503506 Halter fuer NHS KL03:2
- zhu1_XY@8 <-> gba_XY@9 [Mate]: SCHUNK---Grundbacke PGN-plus-P 160-2-P:1 ↔ SCHUNK-9951430 Zentrierhuelse PGN-plus:1
- zhu1_Z@8 <-> gba_Z@9 [Mate]: SCHUNK---Grundbacke PGN-plus-P 160-2-P:1 ↔ SCHUNK-9951430 Zentrierhuelse PGN-plus:1
- zhu1_YZ@8 <-> gba_YZ@9 [Angle] (0 deg): SCHUNK---Grundbacke PGN-plus-P 160-2-P:1 ↔ SCHUNK-9951430 Zentrierhuelse PGN-plus:1
- zhu2_XY@8 <-> gba_XY@10 [Mate]: SCHUNK---Grundbacke PGN-plus-P 160-2-P:1 ↔ SCHUNK-9951430 Zentrierhuelse PGN-plus:2
- zhu2_Z@8 <-> gba_Z@10 [Mate]: SCHUNK---Grundbacke PGN-plus-P 160-2-P:1 ↔ SCHUNK-9951430 Zentrierhuelse PGN-plus:2
- zhu2_YZ@8 <-> gba_YZ@10 [Angle] (0 deg): SCHUNK---Grundbacke PGN-plus-P 160-2-P:1 ↔ SCHUNK-9951430 Zentrierhuelse PGN-plus:2
- zhu1_XY@11 <-> gba_XY@12 [Mate]: SCHUNK---Grundbacke PGN-plus-P 160-2-P:2 ↔ SCHUNK-9951430 Zentrierhuelse PGN-plus:3
- zhu1_Z@11 <-> gba_Z@12 [Mate]: SCHUNK---Grundbacke PGN-plus-P 160-2-P:2 ↔ SCHUNK-9951430 Zentrierhuelse PGN-plus:3
- zhu1_YZ@11 <-> gba_YZ@12 [Angle] (0 deg): SCHUNK---Grundbacke PGN-plus-P 160-2-P:2 ↔ SCHUNK-9951430 Zentrierhuelse PGN-plus:3
- zhu2_XY@11 <-> gba_XY@13 [Mate]: SCHUNK---Grundbacke PGN-plus-P 160-2-P:2 ↔ SCHUNK-9951430 Zentrierhuelse PGN-plus:4
- zhu2_Z@11 <-> gba_Z@13 [Mate]: SCHUNK---Grundbacke PGN-plus-P 160-2-P:2 ↔ SCHUNK-9951430 Zentrierhuelse PGN-plus:4
- zhu2_YZ@11 <-> gba_YZ@13 [Angle] (0 deg): SCHUNK---Grundbacke PGN-plus-P 160-2-P:2 ↔ SCHUNK-9951430 Zentrierhuelse PGN-plus:4
- IP_ALU_XY@14 <-> aluschild_XY@15 [Mate]: FGR AL-2-PGN-plus-P 160,PGN-plus-P 160-2-AS-P81110452001216049_51650000000000000000Aluminium6_5:1 ↔ SCHUNK-9954530 Typenschild 6x17x0_3:1
- IP_ALU_Z@14 <-> aluschild_Z@15 [Mate]: FGR AL-2-PGN-plus-P 160,PGN-plus-P 160-2-AS-P81110452001216049_51650000000000000000Aluminium6_5:1 ↔ SCHUNK-9954530 Typenschild 6x17x0_3:1
- IP_ALU_YZ@14 <-> aluschild_YZ@15 [Angle] (0 deg): FGR AL-2-PGN-plus-P 160,PGN-plus-P 160-2-AS-P81110452001216049_51650000000000000000Aluminium6_5:1 ↔ SCHUNK-9954530 Typenschild 6x17x0_3:1
- IP_SCH_1_XY@14 <-> IP1_XY@16 [Mate]: FGR AL-2-PGN-plus-P 160,PGN-plus-P 160-2-AS-P81110452001216049_51650000000000000000Aluminium6_5:1 ↔ Slotted head cap screw ISO 4762 - M10x35:1
- IP_SCH_1_Z@14 <-> IP1_Z@16 [Mate]: FGR AL-2-PGN-plus-P 160,PGN-plus-P 160-2-AS-P81110452001216049_51650000000000000000Aluminium6_5:1 ↔ Slotted head cap screw ISO 4762 - M10x35:1
- IP_SCH_1_YZ@14 <-> IP1_YZ@16 [Angle] (0 deg): FGR AL-2-PGN-plus-P 160,PGN-plus-P 160-2-AS-P81110452001216049_51650000000000000000Aluminium6_5:1 ↔ Slotted head cap screw ISO 4762 - M10x35:1
- IP_SCH_2_XY@14 <-> IP1_XY@17 [Mate]: FGR AL-2-PGN-plus-P 160,PGN-plus-P 160-2-AS-P81110452001216049_51650000000000000000Aluminium6_5:1 ↔ Slotted head cap screw ISO 4762 - M10x35:2
- IP_SCH_2_Z@14 <-> IP1_Z@17 [Mate]: FGR AL-2-PGN-plus-P 160,PGN-plus-P 160-2-AS-P81110452001216049_51650000000000000000Aluminium6_5:1 ↔ Slotted head cap screw ISO 4762 - M10x35:2
- IP_SCH_2_YZ@14 <-> IP1_YZ@17 [Angle] (0 deg): FGR AL-2-PGN-plus-P 160,PGN-plus-P 160-2-AS-P81110452001216049_51650000000000000000Aluminium6_5:1 ↔ Slotted head cap screw ISO 4762 - M10x35:2
- IP_ALU_XY@18 <-> aluschild_XY@19 [Mate]: FGR AL-2-PGN-plus-P 160,PGN-plus-P 160-2-AS-P81110452001216049_51650000000000000000Aluminium6_5:2 ↔ SCHUNK-9954530 Typenschild 6x17x0_3:2
- IP_ALU_Z@18 <-> aluschild_Z@19 [Mate]: FGR AL-2-PGN-plus-P 160,PGN-plus-P 160-2-AS-P81110452001216049_51650000000000000000Aluminium6_5:2 ↔ SCHUNK-9954530 Typenschild 6x17x0_3:2
- IP_ALU_YZ@18 <-> aluschild_YZ@19 [Angle] (0 deg): FGR AL-2-PGN-plus-P 160,PGN-plus-P 160-2-AS-P81110452001216049_51650000000000000000Aluminium6_5:2 ↔ SCHUNK-9954530 Typenschild 6x17x0_3:2
- IP_SCH_1_XY@18 <-> IP1_XY@20 [Mate]: FGR AL-2-PGN-plus-P 160,PGN-plus-P 160-2-AS-P81110452001216049_51650000000000000000Aluminium6_5:2 ↔ Slotted head cap screw ISO 4762 - M10x35:3
- IP_SCH_1_Z@18 <-> IP1_Z@20 [Mate]: FGR AL-2-PGN-plus-P 160,PGN-plus-P 160-2-AS-P81110452001216049_51650000000000000000Aluminium6_5:2 ↔ Slotted head cap screw ISO 4762 - M10x35:3
- IP_SCH_1_YZ@18 <-> IP1_YZ@20 [Angle] (0 deg): FGR AL-2-PGN-plus-P 160,PGN-plus-P 160-2-AS-P81110452001216049_51650000000000000000Aluminium6_5:2 ↔ Slotted head cap screw ISO 4762 - M10x35:3
- IP_SCH_2_XY@18 <-> IP1_XY@21 [Mate]: FGR AL-2-PGN-plus-P 160,PGN-plus-P 160-2-AS-P81110452001216049_51650000000000000000Aluminium6_5:2 ↔ Slotted head cap screw ISO 4762 - M10x35:4
- IP_SCH_2_Z@18 <-> IP1_Z@21 [Mate]: FGR AL-2-PGN-plus-P 160,PGN-plus-P 160-2-AS-P81110452001216049_51650000000000000000Aluminium6_5:2 ↔ Slotted head cap screw ISO 4762 - M10x35:4
- IP_SCH_2_YZ@18 <-> IP1_YZ@21 [Angle] (0 deg): FGR AL-2-PGN-plus-P 160,PGN-plus-P 160-2-AS-P81110452001216049_51650000000000000000Aluminium6_5:2 ↔ Slotted head cap screw ISO 4762 - M10x35:4
